# Autodesk Inventor assembly: Сборка1
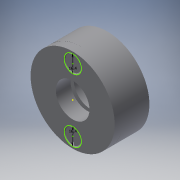
[picture p0: Inventor's stored thumbnail of the model, 180x180]
Saved by Autodesk Inventor 2018 (Build 220112000, 112)
## iProperties
Created: 2018-05-24
Part Number: Сборка1
Material: Типовые
Document SubType Name: Assembly
Designer: user
Author: user
## Documents named in this file (4)
- C:\Users\user\Desktop\Сборка1.iam
- C:\Users\user\Desktop\Корпус.ipt
- C:\Users\user\Desktop\крышка.ipt
- C:\Users\user\Desktop\винт.ipt
## Components (5 placed, 3 different names)
1. Корпус:1 — С поворотом:1, Цилиндрический:1, Цилиндрический:2
2. крышка:1 — С поворотом:1
3. винт:1
4. винт:2 — Цилиндрический:1
5. винт:3 — Цилиндрический:2
## Relationships (3: CylindricalJoint 2, RevoluteJoint 1)
- С поворотом:1 [RevoluteJoint]: Корпус:1 ↔ крышка:1
- Цилиндрический:1 [CylindricalJoint]: Корпус:1 ↔ винт:2
- Цилиндрический:2 [CylindricalJoint]: Корпус:1 ↔ винт:3
